# Autodesk Inventor assembly: Piston_Assembly
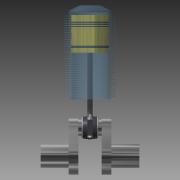
[picture p0: Inventor's stored thumbnail of the model, 180x180]
Saved by Autodesk Inventor 2015 (Build 190159000, 159)
## iProperties
Created: 2021-03-23
Part Number: Piston_Assembly
Document SubType Name: Assembly
Designer: Diptanshu Das
Author: Diptanshu Das
## Documents named in this file (13)
- D:\Entraco_workspace\3D\Animation\Engine Piston\Engine Piston\1L\Piston_Assembly.iam
- D:\Entraco_workspace\3D\Animation\Engine Piston\Engine Piston\1L\bush big end.ipt
- D:\Entraco_workspace\3D\Animation\Engine Piston\Engine Piston\1L\circlip.ipt
- D:\Entraco_workspace\3D\Animation\Engine Piston\Engine Piston\1L\connecting rod.ipt
- D:\Entraco_workspace\3D\Animation\Engine Piston\Engine Piston\1L\end cap.ipt
- D:\Entraco_workspace\3D\Animation\Engine Piston\Engine Piston\1L\piston pin.ipt
- D:\Entraco_workspace\3D\Animation\Engine Piston\Engine Piston\1L\piston.ipt
- D:\Entraco_workspace\3D\Animation\Engine Piston\Engine Piston\1L\Hardwares\hexagon nut style 1_is_IS 1364-3 - M6-D-S.ipt
- D:\Entraco_workspace\3D\Animation\Engine Piston\Engine Piston\1L\Hardwares\hhb(grade a)_is_IS 1364 HHB(Grade A) - M6 x 45 x 18-S.ipt
- D:\Entraco_workspace\3D\Animation\Engine Piston\Engine Piston\1L\crankshaft.ipt
- D:\Entraco_workspace\3D\Animation\Engine Piston\Engine Piston\1L\washer.ipt
- D:\Entraco_workspace\3D\Animation\Engine Piston\Engine Piston\1L\engine block.ipt
- D:\Entraco_workspace\3D\Animation\Engine Piston\Engine Piston\1L\washer 2.ipt
## Components (18 placed, 12 different names)
1. bush big end:1 — Mate:1, Flush:1, Mate:2, Mate:25, Mate:26
2. circlip:1 — Mate:11, Mate:12
3. connecting rod:1 — Mate:1, Flush:1, Mate:2, Mate:5, Mate:6, Mate:7, Mate:8, Flush:3, Mate:10, Mate:18, Mate:22
4. end cap:1 — Mate:3, Flush:2, Mate:4, Mate:5, Mate:6, Mate:7, Mate:15, Mate:16, Mate:20, Mate:21
5. piston pin:1 — Mate:8, Flush:3, Mate:9, Mate:11, Mate:13
6. piston:1 — Mate:9, Mate:10, Mate:12, Mate:14, Mate:23, Mate:24, Mate:28, Mate:29, Mate:30, Mate:31, Mate:32, Mate:33, Mate:34, Mate:35, Mate:36
7. bush big end:2 — Mate:3, Flush:2, Mate:4
8. circlip:2 — Mate:13, Mate:14
9. hexagon nut style 1_is_IS 1364-3 - M6-D-S:1 — Mate:17, Mate:18
10. hhb(grade a)_is_IS 1364 HHB(Grade A) - M6 x 45 x 18-S:1 — Mate:15, Mate:16, Mate:17
11. hexagon nut style 1_is_IS 1364-3 - M6-D-S:2 — Mate:22
12. hhb(grade a)_is_IS 1364 HHB(Grade A) - M6 x 45 x 18-S:2 — Mate:20, Mate:21
13. crankshaft:1 — Mate:25, Mate:26, Mate:27, Angle:1
14. washer:1 — Mate:28, Mate:29
15. washer:2 — Mate:30, Mate:31
16. washer:3 — Mate:32, Mate:33
17. engine block:1 — Mate:34, Flush:4
18. washer 2:1 — Mate:35, Mate:36
## Relationships (41: Mate 36, Flush 4, Angle 1)
- Mate:1: bush big end:1 ↔ connecting rod:1
- Flush:1: bush big end:1 ↔ connecting rod:1
- Mate:2: bush big end:1 ↔ connecting rod:1
- Mate:3: end cap:1 ↔ bush big end:2
- Flush:2: end cap:1 ↔ bush big end:2
- Mate:4: end cap:1 ↔ bush big end:2
- Mate:5: connecting rod:1 ↔ end cap:1
- Mate:6: connecting rod:1 ↔ end cap:1
- Mate:7: connecting rod:1 ↔ end cap:1
- Mate:8: connecting rod:1 ↔ piston pin:1
- Flush:3 (22.5 mm): connecting rod:1 ↔ piston pin:1
- Mate:9: piston pin:1 ↔ piston:1
- Mate:10 (1 mm): connecting rod:1 ↔ piston:1
- Mate:11: circlip:1 ↔ piston pin:1
- Mate:12: circlip:1 ↔ piston:1
- Mate:13: piston pin:1 ↔ circlip:2
- Mate:14: piston:1 ↔ circlip:2
- Mate:15: end cap:1 ↔ hhb(grade a)_is_IS 1364 HHB(Grade A) - M6 x 45 x 18-S:1
- Mate:16: end cap:1 ↔ hhb(grade a)_is_IS 1364 HHB(Grade A) - M6 x 45 x 18-S:1
- Mate:17: hexagon nut style 1_is_IS 1364-3 - M6-D-S:1 ↔ hhb(grade a)_is_IS 1364 HHB(Grade A) - M6 x 45 x 18-S:1
- Mate:18: connecting rod:1 ↔ hexagon nut style 1_is_IS 1364-3 - M6-D-S:1
- [Mate]: hexagon nut style 1_is_IS 1364-3 - M6-D-S:2 ↔ hhb(grade a)_is_IS 1364 HHB(Grade A) - M6 x 45 x 18-S:2
- Mate:20: end cap:1 ↔ hhb(grade a)_is_IS 1364 HHB(Grade A) - M6 x 45 x 18-S:2
- Mate:21: end cap:1 ↔ hhb(grade a)_is_IS 1364 HHB(Grade A) - M6 x 45 x 18-S:2
- Mate:22: connecting rod:1 ↔ hexagon nut style 1_is_IS 1364-3 - M6-D-S:2
- Mate:23: piston:1
- Mate:24: piston:1
- Mate:25: bush big end:1 ↔ crankshaft:1
- Mate:26 (7 mm): bush big end:1 ↔ crankshaft:1
- Mate:27: crankshaft:1
- Angle:1 (180 deg): crankshaft:1
- Mate:28: piston:1 ↔ washer:1
- Mate:29: piston:1 ↔ washer:1
- Mate:30: piston:1 ↔ washer:2
- Mate:31: piston:1 ↔ washer:2
- Mate:32: piston:1 ↔ washer:3
- Mate:33: piston:1 ↔ washer:3
- Mate:34: piston:1 ↔ engine block:1
- Flush:4 (-120 mm): engine block:1
- Mate:35: piston:1 ↔ washer 2:1
- Mate:36: piston:1 ↔ washer 2:1
## Named parameters: d23_d21 = 0 mm
